# Autodesk Inventor assembly: RadioWithMount
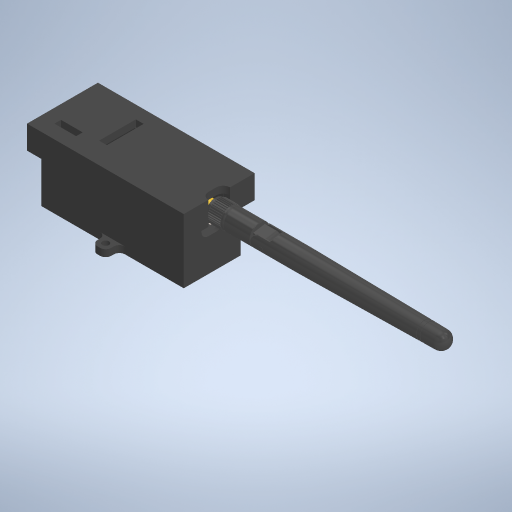
[picture p0: Inventor's stored thumbnail of the model, 512x512]
Saved by Autodesk Inventor 2024 (Build 280153000, 153)
## iProperties
Created: 2023-08-23
Part Number: RadioWithMount
Document SubType Name: Assembly
Designer: 18179
Author: 18179
## Documents named in this file (4)
- C:\Users\18179\Desktop\TuppyMkIV_GitHub\TuppyMkIV\CAD\RadioWithMount.iam
- C:\Users\18179\Desktop\TuppyMkIV_GitHub\TuppyMkIV\CAD\NRF24L01L+Antenna\NRF24L01L+Antenna.iam
- C:\Users\18179\Desktop\TuppyMkIV_GitHub\TuppyMkIV\CAD\RadioMount.ipt
- C:\Users\18179\Desktop\TuppyMkIV_GitHub\TuppyMkIV\CAD\RadioMountCover.ipt
## Components (3 placed, 3 different names)
1. NRF24L01L+Antenna:1 [sub-assembly] — Mate:1, Mate:2, Mate:3
2. RadioMount:1 — Mate:1, Mate:2, Mate:3, Mate:4, Mate:5, Mate:6
3. RadioMountCover:1 — Mate:4, Mate:5, Mate:6
## Relationships (6: Mate 6)
- Mate:1 (1 mm): NRF24L01L+Antenna:1 ↔ RadioMount:1
- Mate:2 (1 mm): NRF24L01L+Antenna:1 ↔ RadioMount:1
- Mate:3: NRF24L01L+Antenna:1 ↔ RadioMount:1
- Mate:4: RadioMount:1 ↔ RadioMountCover:1
- Mate:5: RadioMount:1 ↔ RadioMountCover:1
- Mate:6: RadioMount:1 ↔ RadioMountCover:1
